# Autodesk Inventor assembly: YagiBoard
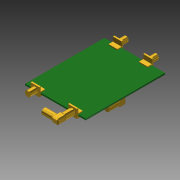
[picture p0: Inventor's stored thumbnail of the model, 180x180]
Saved by Autodesk Inventor 2014 (Build 180170000, 170)
## iProperties
Created: 2015-01-07
Part Number: YagiBoard
Document SubType Name: Assembly
Designer: Owner
Author: Owner
## Documents named in this file (5)
- C:\Users\Owner\Documents\APC\FrontEnd\IAM\Yagi\YagiBoard.iam
- C:\Users\Owner\Documents\APC\FrontEnd\IAM\Yagi\Yagi_Board.ipt
- C:\Users\Owner\Documents\APC\FrontEnd\IAM\Common\SMA_Edge.ipt
- C:\Users\Owner\Documents\APC\FrontEnd\IAM\Common\SMA_RightAngle.ipt
- C:\Users\Owner\Documents\APC\FrontEnd\IAM\Common\SMA_Up.ipt
## Components (8 placed, 4 different names)
1. Yagi_Board:1 — Mate:1, Mate:2, Mate:3, Mate:4, Mate:5, Mate:6, Mate:7, Mate:8, Flush:1, Flush:2, Mate:17, Flush:3, Flush:4
2. SMA_Edge:1 — Mate:3, Mate:6, Flush:1
3. SMA_Edge:2 — Mate:2, Mate:7, Flush:2
4. SMA_Edge:3 — Mate:4, Mate:5, Flush:3, Mate:20, Mate:21
5. SMA_Edge:4 — Mate:1, Mate:8, Flush:4
6. SMA_Up:1 — Mate:17, Mate:18, Mate:19
7. SMA_RightAngle:5 — Mate:18, Mate:19
8. SMA_RightAngle:6 — Mate:20, Mate:21
## Relationships (17: Mate 13, Flush 4)
- Mate:1: Yagi_Board:1 ↔ SMA_Edge:4
- Mate:2: Yagi_Board:1 ↔ SMA_Edge:2
- Mate:3: Yagi_Board:1 ↔ SMA_Edge:1
- Mate:4: Yagi_Board:1 ↔ SMA_Edge:3
- Mate:5: Yagi_Board:1 ↔ SMA_Edge:3
- Mate:6: Yagi_Board:1 ↔ SMA_Edge:1
- Mate:7: Yagi_Board:1 ↔ SMA_Edge:2
- Mate:8: Yagi_Board:1 ↔ SMA_Edge:4
- Flush:1 (-9.2202 mm): Yagi_Board:1 ↔ SMA_Edge:1
- Flush:2 (14.478 mm): Yagi_Board:1 ↔ SMA_Edge:2
- Mate:17: Yagi_Board:1 ↔ SMA_Up:1
- Mate:18: SMA_Up:1 ↔ SMA_RightAngle:5
- Mate:19 (2 mm): SMA_Up:1 ↔ SMA_RightAngle:5
- Flush:3 (8.128 mm): Yagi_Board:1 ↔ SMA_Edge:3
- Flush:4 (7.62 mm): Yagi_Board:1 ↔ SMA_Edge:4
- Mate:20: SMA_Edge:3 ↔ SMA_RightAngle:6
- Mate:21 (2 mm): SMA_Edge:3 ↔ SMA_RightAngle:6
